# Autodesk Inventor assembly: Load_Cell_Hopper_Connection
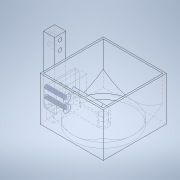
[picture p0: Inventor's stored thumbnail of the model, 180x180]
Saved by Autodesk Inventor 2022 (Build 260153000, 153)
## iProperties
Created: 2022-09-14
Part Number: Load_Cell_Hopper_Connection
Document SubType Name: Assembly
Designer: tecssupport
Author: tecssupport
## Documents named in this file (5)
- E:\College Stuff\ATMAE Robotics\Pill Dispenser Robot\Load Cell_Hopper_Connection\Load_Cell_Hopper_Connection.iam
- E:\College Stuff\ATMAE Robotics\Pill Dispenser Robot\Load Cell_Hopper_Connection\Traingular Hopper Connector.ipt
- E:\College Stuff\ATMAE Robotics\Pill Dispenser Robot\Load Cell_Hopper_Connection\Load_Cell.ipt
- E:\College Stuff\ATMAE Robotics\Pill Dispenser Robot\Hoppers\M&M Hopper\main Hopper body v6.ipt
- E:\College Stuff\ATMAE Robotics\Pill Dispenser Robot\Load Cell_Hopper_Connection\M4 25mm Length Flat Head Screw.ipt
## Components (5 placed, 4 different names)
1. Load_Cell:1 — Mate:1, Mate:2, Mate:3, Mate:8
2. main Hopper body v6:1 — Mate:4, Mate:5, Mate:6
3. Traingular Hopper Connector:1 — Mate:1, Mate:2, Mate:3, Mate:4, Mate:5, Mate:6, Mate:7, Flush:1, Flush:2
4. M4 25mm Length Flat Head Screw:1 — Mate:8, Flush:2
5. M4 25mm Length Flat Head Screw:2 — Mate:7, Flush:1
## Relationships (10: Mate 8, Flush 2)
- Mate:1: Load_Cell:1 ↔ Traingular Hopper Connector:1
- Mate:2: Load_Cell:1 ↔ Traingular Hopper Connector:1
- Mate:3: Load_Cell:1 ↔ Traingular Hopper Connector:1
- Mate:4: main Hopper body v6:1 ↔ Traingular Hopper Connector:1
- Mate:5: main Hopper body v6:1 ↔ Traingular Hopper Connector:1
- Mate:6: main Hopper body v6:1 ↔ Traingular Hopper Connector:1
- Mate:7: Traingular Hopper Connector:1 ↔ M4 25mm Length Flat Head Screw:2
- Flush:1: Traingular Hopper Connector:1 ↔ M4 25mm Length Flat Head Screw:2
- Mate:8: Load_Cell:1 ↔ M4 25mm Length Flat Head Screw:1
- Flush:2: Traingular Hopper Connector:1 ↔ M4 25mm Length Flat Head Screw:1
